# Autodesk Inventor assembly: axis5_6
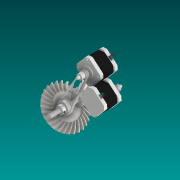
[picture p0: Inventor's stored thumbnail of the model, 180x180]
Saved by Autodesk Inventor 2020 (Build 240168000, 168)
## iProperties
Created: 2020-05-15
Part Number: axis5_6
Document SubType Name: Assembly
Designer: stefa
Author: stefa
## Documents named in this file (7)
- D:\github_gedeeld\BeerMinder\3D-model\axis5_6\axis5_6.iam
- D:\github_gedeeld\BeerMinder\3D-model\pulleys\tandriem32Tnaar16T_lengte240.ipt
- D:\github_gedeeld\BeerMinder\3D-model\pulleys\GT2 Timing Pulley 36T - 8mm as.ipt
- D:\github_gedeeld\BeerMinder\3D-model\stepper motors\42BYG Stepper Motor.ipt
- D:\github_gedeeld\BeerMinder\3D-model\pulleys\GT2 Pulley 16T - 5mm as.ipt
- D:\github_gedeeld\BeerMinder\3D-model\axis5_6\as_d8_l100.ipt
- D:\github_gedeeld\BeerMinder\3D-model\axis5_6\axis5_6\Design Accelerator\Bevel Gears1.iam
## Components (10 placed, 6 different names)
1. tandriem32Tnaar16T_lengte240:1 — Mate:5, Mate:6, Mate:21, Mate:22
2. GT2 Pulley 16T - 5mm as:1 — Mate:5, Mate:6, Mate:15, Mate:16
3. as_d8_l100:1 — Mate:20, Mate:23, Mate:26
4. tandriem32Tnaar16T_lengte240:2 — Mate:24, Mate:25
5. GT2 Pulley 16T - 5mm as:2 — Mate:17, Mate:18
6. Bevel Gears:1 [sub-assembly] — Mate:26
7. 42BYG Stepper Motor:2 — Mate:15, Mate:16, Flush:1, Mate:19, Flush:2
8. 42BYG Stepper Motor:3 — Mate:17, Mate:18, Flush:1, Mate:19, Flush:2
9. GT2 Timing Pulley 36T - 8mm as:3 — Mate:23, Mate:24, Mate:25
10. GT2 Timing Pulley 36T - 8mm as:4 — Mate:20, Mate:21, Mate:22
## Relationships (18: Mate 16, Flush 2)
- Mate:5: tandriem32Tnaar16T_lengte240:1 ↔ GT2 Pulley 16T - 5mm as:1
- Mate:6 (0.5 mm): tandriem32Tnaar16T_lengte240:1 ↔ GT2 Pulley 16T - 5mm as:1
- [Mate]: tandriem32Tnaar16T_lengte240:2 ↔ GT2 Pulley 16T - 5mm as:2
- [Mate] (0.5 mm): tandriem32Tnaar16T_lengte240:2 ↔ GT2 Pulley 16T - 5mm as:2
- Mate:15: GT2 Pulley 16T - 5mm as:1 ↔ 42BYG Stepper Motor:2
- Mate:16 (2 mm): GT2 Pulley 16T - 5mm as:1 ↔ 42BYG Stepper Motor:2
- Mate:17 (2 mm): GT2 Pulley 16T - 5mm as:2 ↔ 42BYG Stepper Motor:3
- Mate:18: GT2 Pulley 16T - 5mm as:2 ↔ 42BYG Stepper Motor:3
- Flush:1: 42BYG Stepper Motor:2 ↔ 42BYG Stepper Motor:3
- Mate:19 (2 mm): 42BYG Stepper Motor:2 ↔ 42BYG Stepper Motor:3
- Flush:2: 42BYG Stepper Motor:2 ↔ 42BYG Stepper Motor:3
- Mate:20: as_d8_l100:1 ↔ GT2 Timing Pulley 36T - 8mm as:4
- Mate:21: tandriem32Tnaar16T_lengte240:1 ↔ GT2 Timing Pulley 36T - 8mm as:4
- Mate:22 (0.5 mm): tandriem32Tnaar16T_lengte240:1 ↔ GT2 Timing Pulley 36T - 8mm as:4
- Mate:23: as_d8_l100:1 ↔ GT2 Timing Pulley 36T - 8mm as:3
- Mate:24: tandriem32Tnaar16T_lengte240:2 ↔ GT2 Timing Pulley 36T - 8mm as:3
- Mate:25 (0.5 mm): tandriem32Tnaar16T_lengte240:2 ↔ GT2 Timing Pulley 36T - 8mm as:3
- Mate:26: as_d8_l100:1 ↔ Bevel Gears:1
## Named parameters: d13_d6 = 0 mm, d14_d7 = 0.5 mm
